# Autodesk Inventor assembly: Assembly4
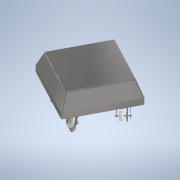
[picture p0: Inventor's stored thumbnail of the model, 180x180]
Saved by Autodesk Inventor 2020 (Build 240168000, 168)
## iProperties
Created: 2022-06-28
Part Number: Assembly4
Document SubType Name: Assembly
Designer: karimi2
Author: karimi2
## Documents named in this file (4)
- C:\Users\karimi2\Documents\PROJECT\Assembly4.iam
- C:\Users\karimi2\Documents\PROJECT\Body.ipt
- C:\Users\karimi2\Documents\PROJECT\Assembly4\Design Accelerator\Bearing1.iam
- C:\Users\karimi2\Documents\PROJECT\Assembly2.iam
## Components (9 placed, 3 different names)
1. Body:1 — Mate:1, Flush:1, Mate:2, Flush:2, Mate:3, Flush:3, Mate:4, Flush:4
2. Bearing:1 [sub-assembly] — Mate:4, Flush:4, Mate:7, Mate:8
3. Bearing:3 [sub-assembly] — Mate:2, Flush:2, Mate:11, Mate:12
4. Bearing:4 [sub-assembly] — Mate:1, Flush:1, Mate:5, Mate:6
5. Bearing:5 [sub-assembly] — Mate:3, Flush:3, Mate:9, Mate:10
6. Assembly2:1 [sub-assembly] — Mate:5, Mate:6
7. Assembly2:2 [sub-assembly] — Mate:9, Mate:10
8. Assembly2:3 [sub-assembly] — Mate:11, Mate:12
9. Assembly2:4 [sub-assembly] — Mate:7, Mate:8
## Relationships (16: Mate 12, Flush 4)
- Mate:1: Body:1 ↔ Bearing:4
- Flush:1 (-4.5 mm): Body:1 ↔ Bearing:4
- Mate:2: Body:1 ↔ Bearing:3
- Flush:2 (-4.5 mm): Body:1 ↔ Bearing:3
- Mate:3: Body:1 ↔ Bearing:5
- Flush:3 (-4.5 mm): Body:1 ↔ Bearing:5
- Mate:4: Body:1 ↔ Bearing:1
- Flush:4 (-4.5 mm): Body:1 ↔ Bearing:1
- Mate:5: Bearing:4 ↔ Assembly2:1
- Mate:6 (4 mm): Bearing:4 ↔ Assembly2:1
- Mate:7: Bearing:1 ↔ Assembly2:4
- Mate:8 (4 mm): Bearing:1 ↔ Assembly2:4
- Mate:9: Bearing:5 ↔ Assembly2:2
- Mate:10 (4 mm): Bearing:5 ↔ Assembly2:2
- Mate:11: Bearing:3 ↔ Assembly2:3
- Mate:12 (4 mm): Bearing:3 ↔ Assembly2:3
